# Autodesk Inventor assembly: DroneSet
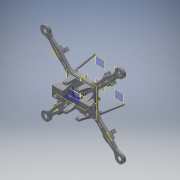
[picture p0: Inventor's stored thumbnail of the model, 180x180]
Saved by Autodesk Inventor 2019 (Build 230136000, 136)
## iProperties
Created: 2018-09-18
Part Number: DroneSet
Material: Generico
Document SubType Name: Assembly
Designer: acorbeau
Author: acorbeau
## Documents named in this file (16)
- C:\Users\acorbeau\Documents\DroneX\DroneSet.iam
- C:\Users\acorbeau\Documents\DroneX\DroneBase.ipt
- C:\Users\acorbeau\Documents\DroneX\Pièce5.ipt
- C:\Users\acorbeau\Documents\DroneX\Brace.ipt
- C:\Users\acorbeau\Documents\DroneX\LandingPad.ipt
- C:\Users\acorbeau\Documents\DroneX\Brace_MIR.ipt
- C:\Users\acorbeau\Documents\DroneX\LandingPad_MIR.ipt
- C:\Users\acorbeau\Documents\DroneX\Brace_MIR1.ipt
- C:\Users\acorbeau\Documents\DroneX\LandingPad_MIR1.ipt
- C:\Users\acorbeau\Documents\DroneX\Brace_MIR_MIR.ipt
- C:\Users\acorbeau\Documents\DroneX\LandingPad_MIR_MIR.ipt
- C:\Users\acorbeau\Documents\DroneX\ServoSuport.ipt
- C:\Users\acorbeau\Documents\DroneX\ESCFixation.ipt
- C:\Users\acorbeau\Documents\DroneX\ESCFixation_MIR.ipt
- C:\Users\acorbeau\Documents\DroneX\ESCFixation_MIR1.ipt
- C:\Users\acorbeau\Documents\DroneX\ESCFixation_MIR_MIR.ipt
## Components (15 placed, 15 different names)
1. DroneBase:1 — Placage:1, Placage:2, Placage:8, Affleurement:1, Affleurement:2, Placage:13
2. DroneBaseCap:1 — Placage:1, Placage:2, Placage:10, Placage:11, Placage:12
3. Brace:1 — Placage:8, Placage:10
4. LandingPad:1 — Placage:11, Placage:12
5. Brace_MIR:1
6. LandingPad_MIR:1
7. Brace_MIR1:1
8. LandingPad_MIR1:1
9. Brace_MIR_MIR:1
10. LandingPad_MIR_MIR:1
11. ESCFixation:1
12. ESCFixation_MIR:1
13. ESCFixation_MIR1:1
14. ESCFixation_MIR_MIR:1
15. ServoSuport:1 — Placage:13
## Relationships (9: Mate 7, Flush 2)
- Placage:1 [Mate]: DroneBase:1 ↔ DroneBaseCap:1
- Placage:2 [Mate]: DroneBase:1 ↔ DroneBaseCap:1
- Placage:8 [Mate]: DroneBase:1 ↔ Brace:1
- Placage:10 [Mate]: DroneBaseCap:1 ↔ Brace:1
- Placage:11 [Mate]: DroneBaseCap:1 ↔ LandingPad:1
- Placage:12 [Mate]: DroneBaseCap:1 ↔ LandingPad:1
- Affleurement:1 [Flush] (-40 mm): DroneBase:1
- Affleurement:2 [Flush] (-40 mm): DroneBase:1
- Placage:13 [Mate]: DroneBase:1 ↔ ServoSuport:1
